# Autodesk Inventor assembly: Bird_wing_10_large_V2
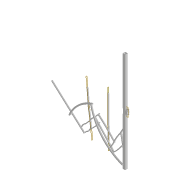
[picture p0: Inventor's stored thumbnail of the model, 180x180]
Saved by Autodesk Inventor 2022 (Build 260153000, 153)
## iProperties
Created: 2022-04-26
Part Number: Bird_wing_10_large_V2
Document SubType Name: Assembly
Designer: dell
Author: dell
## Documents named in this file (15)
- D:\xxxx\Uni\Part IV\MECHENG_700\Part_IV_project_CAD\Bird_skeleton_prototypes\Wing_drone_V1\Bird_wing_10_large_V2.iam
- D:\xxxx\Uni\Part IV\MECHENG_700\Part_IV_project_CAD\Bird_skeleton_prototypes\Wing_drone_V1\Drone_wing_skeleton\Part_2.ipt
- D:\xxxx\Uni\Part IV\MECHENG_700\Part_IV_project_CAD\Bird_skeleton_prototypes\Wing_drone_V1\Drone_wing_skeleton\Part_4.ipt
- D:\xxxx\Uni\Part IV\MECHENG_700\Part_IV_project_CAD\Bird_skeleton_prototypes\Wing_drone_V1\Drone_wing_skeleton\Part_3.ipt
- D:\xxxx\Uni\Part IV\MECHENG_700\Part_IV_project_CAD\Bird_skeleton_prototypes\Wing_drone_V1\Drone_wing_skeleton\Part_16.ipt
- D:\xxxx\Uni\Part IV\MECHENG_700\Part_IV_project_CAD\Bird_skeleton_prototypes\Wing_drone_V1\Drone_wing_skeleton\Part_5.ipt
- D:\xxxx\Uni\Part IV\MECHENG_700\Part_IV_project_CAD\Bird_skeleton_prototypes\Wing_drone_V1\Drone_wing_skeleton\Part_7.ipt
- D:\xxxx\Uni\Part IV\MECHENG_700\Part_IV_project_CAD\Bird_skeleton_prototypes\Wing_drone_V1\Drone_wing_skeleton\Part_9.ipt
- D:\xxxx\Uni\Part IV\MECHENG_700\Part_IV_project_CAD\Bird_skeleton_prototypes\Wing_drone_V1\Drone_wing_skeleton\Part_10.ipt
- D:\xxxx\Uni\Part IV\MECHENG_700\Part_IV_project_CAD\Bird_skeleton_prototypes\Wing_drone_V1\Drone_wing_skeleton\Part_13.ipt
- D:\xxxx\Uni\Part IV\MECHENG_700\Part_IV_project_CAD\Bird_skeleton_prototypes\Wing_drone_V1\Drone_wing_skeleton\Part_12.ipt
- D:\xxxx\Uni\Part IV\MECHENG_700\Part_IV_project_CAD\Bird_skeleton_prototypes\Wing_drone_V1\Drone_wing_skeleton\Part_8.ipt
- D:\xxxx\Uni\Part IV\MECHENG_700\Part_IV_project_CAD\Bird_skeleton_prototypes\Wing_drone_V1\Drone_wing_skeleton\Part_11.ipt
- D:\xxxx\Uni\Part IV\MECHENG_700\Part_IV_project_CAD\Bird_skeleton_prototypes\Wing_drone_V1\Square_tube_connector.ipt
- D:\xxxx\Uni\Part IV\MECHENG_700\Part_IV_project_CAD\Bird_skeleton_prototypes\Wing_drone_V1\Square_tube_arm.ipt
## Components (15 placed, 14 different names)
1. Part_2:1 — Mate:3, Mate:4, Mate:5, Mate:6
2. Part_4:1 — Mate:3, Mate:4, Mate:8, Mate:9
3. Part_3:1 — Mate:5, Mate:6, Mate:10, Mate:11, Mate:12
4. Part_16:1 — Mate:8, Mate:9, Mate:10, Mate:27, Mate:28, Mate:31, Mate:35, Mate:36
5. Part_5:1 — Mate:11, Mate:12, Mate:32, Mate:33, Mate:37
6. Part_7:1 — Mate:30, Mate:31, Mate:32, Mate:33, Mate:34, Mate:41
7. Part_9:1 — Mate:26, Mate:27, Mate:28, Mate:39, Mate:40
8. Part_10:1 — Mate:21, Mate:22, Mate:26, Mate:30, Mate:34
9. Part_13:1 — Mate:23, Mate:24
10. Part_12:1 — Mate:21, Mate:22, Mate:23, Mate:24
11. Part_8:1 — Mate:35, Mate:36, Mate:37
12. Part_11:1 — Mate:39, Mate:40, Mate:41
13. Square_tube_connector:2 — Mate:42, Mate:43, Mate:44, Mate:45, Mate:46, Mate:47
14. Square_tube_arm:2 — Mate:42, Mate:43, Mate:44
15. Square_tube_arm:3 — Mate:45, Mate:46, Mate:47
## Relationships (33: Mate 33)
- Mate:3: Part_2:1 ↔ Part_4:1
- Mate:4: Part_2:1 ↔ Part_4:1
- Mate:5: Part_2:1 ↔ Part_3:1
- Mate:6: Part_2:1 ↔ Part_3:1
- Mate:8: Part_4:1 ↔ Part_16:1
- Mate:9: Part_4:1 ↔ Part_16:1
- Mate:10: Part_3:1 ↔ Part_16:1
- Mate:11: Part_3:1 ↔ Part_5:1
- Mate:12: Part_3:1 ↔ Part_5:1
- Mate:21: Part_10:1 ↔ Part_12:1
- Mate:22: Part_10:1 ↔ Part_12:1
- Mate:23: Part_13:1 ↔ Part_12:1
- Mate:24: Part_13:1 ↔ Part_12:1
- Mate:26: Part_9:1 ↔ Part_10:1
- Mate:27: Part_16:1 ↔ Part_9:1
- Mate:28: Part_16:1 ↔ Part_9:1
- Mate:30: Part_7:1 ↔ Part_10:1
- Mate:31: Part_16:1 ↔ Part_7:1
- Mate:32: Part_5:1 ↔ Part_7:1
- Mate:33: Part_5:1 ↔ Part_7:1
- Mate:34: Part_7:1 ↔ Part_10:1
- Mate:35: Part_16:1 ↔ Part_8:1
- Mate:36: Part_16:1 ↔ Part_8:1
- Mate:37: Part_5:1 ↔ Part_8:1
- Mate:39: Part_9:1 ↔ Part_11:1
- Mate:40: Part_9:1 ↔ Part_11:1
- Mate:41: Part_7:1 ↔ Part_11:1
- Mate:42 (0.05 mm): Square_tube_connector:2 ↔ Square_tube_arm:2
- Mate:43 (0.05 mm): Square_tube_connector:2 ↔ Square_tube_arm:2
- Mate:44: Square_tube_connector:2 ↔ Square_tube_arm:2
- Mate:45 (0.05 mm): Square_tube_connector:2 ↔ Square_tube_arm:3
- Mate:46 (0.05 mm): Square_tube_connector:2 ↔ Square_tube_arm:3
- Mate:47: Square_tube_connector:2 ↔ Square_tube_arm:3
